# Autodesk Inventor assembly: PcbsAssembly
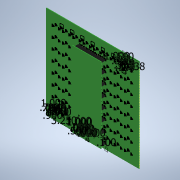
[picture p0: Inventor's stored thumbnail of the model, 180x180]
Saved by Autodesk Inventor 2020 (Build 240168000, 168)
## iProperties
Created: 2020-04-12
Part Number: PcbsAssembly
Document SubType Name: Assembly
Designer: torto
Author: torto
## Documents named in this file (4)
- C:\Users\torto\OneDrive\Documents\Projects\LED Cube\Mechanical\Inventor\PcbsAssembly.iam
- C:\Users\torto\OneDrive\Documents\Projects\LED Cube\Mechanical\Inventor\Cube_Pcb.ipt
- C:\Users\torto\OneDrive\Documents\Projects\LED Cube\Mechanical\Inventor\1x8 SMD Header.ipt
- C:\Users\torto\OneDrive\Documents\Projects\LED Cube\Mechanical\Inventor\DaughterBoard.ipt
## Components (26 placed, 3 different names)
1. Cube_Pcb:1 — Mate:1, Mate:2, Mate:3
2. DaughterBoard:1 — Mate:4, Flush:1, Flush:2
3. 1x8 SMD Header:1 — Mate:1, Mate:2, Mate:3, Mate:4
4. 1x8 SMD Header:2
5. 1x8 SMD Header:3
6. 1x8 SMD Header:4
7. 1x8 SMD Header:5
8. 1x8 SMD Header:6
9. 1x8 SMD Header:7
10. 1x8 SMD Header:8
11. 1x8 SMD Header:9
12. 1x8 SMD Header:10
13. 1x8 SMD Header:11
14. 1x8 SMD Header:12
15. 1x8 SMD Header:13
16. 1x8 SMD Header:14
17. 1x8 SMD Header:15
18. 1x8 SMD Header:16
19. 1x8 SMD Header:17
20. 1x8 SMD Header:18
21. 1x8 SMD Header:19
22. 1x8 SMD Header:20
23. 1x8 SMD Header:21
24. 1x8 SMD Header:22
25. 1x8 SMD Header:23
26. 1x8 SMD Header:24 — Flush:1, Flush:2
## Component patterns: (24 elements, first: 1x8 SMD Header:1)
## Relationships (6: Mate 4, Flush 2)
- Mate:1: Cube_Pcb:1 ↔ 1x8 SMD Header:1
- Mate:2: Cube_Pcb:1 ↔ 1x8 SMD Header:1
- Mate:3: Cube_Pcb:1 ↔ 1x8 SMD Header:1
- Mate:4: DaughterBoard:1 ↔ 1x8 SMD Header:1
- Flush:1: DaughterBoard:1 ↔ 1x8 SMD Header:24
- Flush:2: DaughterBoard:1 ↔ 1x8 SMD Header:24
